# Autodesk Inventor assembly: Torch Holder Assembly V2
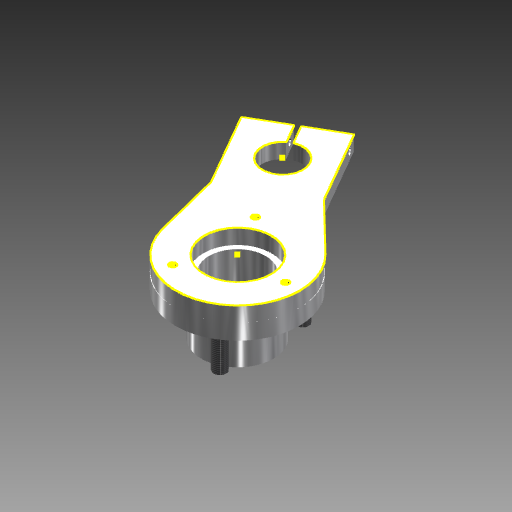
[picture p0: Inventor's stored thumbnail of the model, 512x512]
Saved by Autodesk Inventor 2019 (Build 230136000, 136)
## iProperties
Created: 2018-02-18
Part Number: Torch Holder Assembly V2
Document SubType Name: Assembly
Designer: torba
Author: torba
## Documents named in this file (5)
- C:\Users\torba\OneDrive\Documents\Inventor\Plasma 5x10\Torch Holder Assembly V2.iam
- C:\Users\torba\OneDrive\Documents\Inventor\Plasma 5x10\Torch Holder Base.ipt
- C:\Users\torba\OneDrive\Documents\Inventor\Plasma 5x10\Inductive Sensor NO.ipt
- C:\Users\torba\OneDrive\Documents\Inventor\Plasma 5x10\Torch Holder Upper.ipt
- C:\Users\torba\OneDrive\Documents\Inventor\Content Center Files\R2018\en-US\AS 1420\AS 1420 - 1973 - M5 x 40.ipt
## Components (8 placed, 4 different names)
1. Torch Holder Base:1 — Mate:4, Mate:5, Mate:6, Mate:7, Mate:8, Mate:9, Flush:4, Flush:5, Flush:6
2. Inductive Sensor NO:1 — Mate:1, Flush:1
3. Inductive Sensor NO:2 — Mate:2, Flush:3
4. Inductive Sensor NO:3 — Mate:3, Flush:2
5. Torch Holder Upper:1 — Mate:1, Mate:2, Mate:3, Flush:1, Flush:2, Flush:3, Mate:4, Mate:5, Mate:6
6. AS 1420 - Metric M5 x 40:1 — Mate:7, Flush:5
7. AS 1420 - Metric M5 x 40:2 — Mate:8, Flush:4
8. AS 1420 - Metric M5 x 40:3 — Mate:9, Flush:6
## Relationships (15: Mate 9, Flush 6)
- Mate:1: Inductive Sensor NO:1 ↔ Torch Holder Upper:1
- Mate:2: Inductive Sensor NO:2 ↔ Torch Holder Upper:1
- Mate:3: Inductive Sensor NO:3 ↔ Torch Holder Upper:1
- Flush:1 (2 mm): Inductive Sensor NO:1 ↔ Torch Holder Upper:1
- Flush:2 (2 mm): Inductive Sensor NO:3 ↔ Torch Holder Upper:1
- Flush:3 (2 mm): Inductive Sensor NO:2 ↔ Torch Holder Upper:1
- Mate:4: Torch Holder Base:1 ↔ Torch Holder Upper:1
- Mate:5: Torch Holder Base:1 ↔ Torch Holder Upper:1
- Mate:6: Torch Holder Base:1 ↔ Torch Holder Upper:1
- Mate:7: Torch Holder Base:1 ↔ AS 1420 - Metric M5 x 40:1
- Mate:8: Torch Holder Base:1 ↔ AS 1420 - Metric M5 x 40:2
- Mate:9: Torch Holder Base:1 ↔ AS 1420 - Metric M5 x 40:3
- Flush:4: Torch Holder Base:1 ↔ AS 1420 - Metric M5 x 40:2
- Flush:5: Torch Holder Base:1 ↔ AS 1420 - Metric M5 x 40:1
- Flush:6: Torch Holder Base:1 ↔ AS 1420 - Metric M5 x 40:3
